# Autodesk Inventor assembly: Assembly1
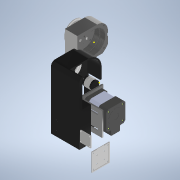
[picture p0: Inventor's stored thumbnail of the model, 180x180]
Saved by Autodesk Inventor 2022 (Build 260153000, 153)
## iProperties
Created: 2022-03-19
Part Number: Assembly1
Document SubType Name: Assembly
Designer: Mlees
Author: Mlees
## Documents named in this file (18)
- C:\Users\Mlees\Desktop\504Engineering\Stepper-Servo_Based_Robotic_Arm\Designs\Documentation_assembly\Assembly1.iam
- C:\Users\Mlees\Desktop\504Engineering\Stepper-Servo_Based_Robotic_Arm\Designs\Version_7\Created_Parts\Combined_Gear_Box_Modified_3.ipt
- C:\Users\Mlees\Desktop\504Engineering\Stepper-Servo_Based_Robotic_Arm\Designs\Version_7\Created_Parts\Metal_AttachmentBracket.ipt
- C:\Users\Mlees\Desktop\504Engineering\Stepper-Servo_Based_Robotic_Arm\Designs\Version_7\Downloaded_Parts\91290A113_Black-Oxide Alloy Steel Socket Head Screw.ipt
- C:\Users\Mlees\Desktop\504Engineering\Stepper-Servo_Based_Robotic_Arm\Designs\Version_7\Downloaded_Parts\nema17-speed-reducer-1.snapshot.9\Thread Insert M3 x 6mm v2.step.iam
- C:\Users\Mlees\Desktop\504Engineering\Stepper-Servo_Based_Robotic_Arm\Designs\Version_7\Downloaded_Parts\124125202-9-stp-mtr-17040w\stp-mtr-17040w.ipt
- C:\Users\Mlees\Desktop\504Engineering\Stepper-Servo_Based_Robotic_Arm\Designs\Version_7\Downloaded_Parts\GT2 20T Drive Pulley.ipt
- C:\Users\Mlees\Desktop\504Engineering\Stepper-Servo_Based_Robotic_Arm\Designs\Version_8\Downloaded_Parts\92010A018_Passivated 18-8 Stainless Steel Phillips Flat Head Screw.ipt
- C:\Users\Mlees\Desktop\504Engineering\Stepper-Servo_Based_Robotic_Arm\Designs\Version_8\Created_Parts\Belt_Bearing_Holder.ipt
- C:\Users\Mlees\Desktop\504Engineering\Stepper-Servo_Based_Robotic_Arm\Designs\Version_8\Created_Parts\Belt_Bearing_Holder_p2.ipt
- C:\Users\Mlees\Desktop\504Engineering\Stepper-Servo_Based_Robotic_Arm\Designs\Version_8\Downloaded_Parts\5972K225_Ball Bearing.ipt
- C:\Users\Mlees\Desktop\504Engineering\Stepper-Servo_Based_Robotic_Arm\Designs\Version_8\Downloaded_Parts\91290A059_Black-Oxide Alloy Steel Socket Head Screw_M3_30mm.ipt
- C:\Users\Mlees\Desktop\504Engineering\Stepper-Servo_Based_Robotic_Arm\Designs\Version_8\Downloaded_Parts\5972K327_Ball Bearing_6201-2Z.ipt
- C:\Users\Mlees\Desktop\504Engineering\Stepper-Servo_Based_Robotic_Arm\Designs\Version_8\Created_Parts\Combined_Gear_Box_Modified_2.ipt
- C:\Users\Mlees\Desktop\504Engineering\Stepper-Servo_Based_Robotic_Arm\Designs\Version_8\Created_Parts\Mag_Shield_Back.ipt
- C:\Users\Mlees\Desktop\504Engineering\Stepper-Servo_Based_Robotic_Arm\Designs\Version_8\Created_Parts\Mag_Sensor.ipt
- C:\Users\Mlees\Desktop\504Engineering\Stepper-Servo_Based_Robotic_Arm\Designs\Version_8\Downloaded_Parts\9403T15_Tight-Tolerance High-Strength 7075 Aluminum Rod.ipt
- C:\Users\Mlees\Desktop\504Engineering\Stepper-Servo_Based_Robotic_Arm\Designs\Version_8\Downloaded_Parts\GT2 60T Drive Pulley.ipt
## Components (29 placed, 17 different names)
1. Combined_Gear_Box_Modified_3:1 — Mate:1, Mate:2, Mate:3, Mate:4, Flush:1, Flush:2, Flush:3, Flush:4, Mate:5, Flush:5, Mate:6, Mate:15, Mate:16, Flush:6, Flush:7, Rotational:2, Rotational:3, Mate:27, Flush:12
2. Metal_AttachmentBracket:1 — Mate:5, Flush:5, Mate:6, Mate:11, Mate:12, Mate:13, Mate:14, Mate:17, Mate:18, Mate:19, Mate:20, Flush:8, Flush:9, Flush:10, Flush:11
3. 91290A113_Black-Oxide Alloy Steel Socket Head Screw:1 — Mate:7, Mate:12
4. 91290A113_Black-Oxide Alloy Steel Socket Head Screw:2 — Mate:8, Mate:11
5. 91290A113_Black-Oxide Alloy Steel Socket Head Screw:3 — Mate:9, Mate:13
6. 91290A113_Black-Oxide Alloy Steel Socket Head Screw:4 — Mate:10, Mate:14
7. Thread Insert M3 x 6mm v2.step:1 [sub-assembly] — Mate:1, Flush:3, Mate:8
8. Thread Insert M3 x 6mm v2.step:2 [sub-assembly] — Mate:4, Flush:1, Mate:9
9. Thread Insert M3 x 6mm v2.step:3 [sub-assembly] — Mate:3, Flush:4, Mate:10
10. Thread Insert M3 x 6mm v2.step:4 [sub-assembly] — Mate:2, Flush:2, Mate:7
11. Thread Insert M3 x 6mm v2.step:5 [sub-assembly] — Mate:15, Flush:6
12. Thread Insert M3 x 6mm v2.step:6 [sub-assembly] — Mate:16, Flush:7
13. stp-mtr-17040w:1 — Rotational:1
14. GT2 20T Drive Pulley:1 — Rotational:1
15. 92010A018_Passivated 18-8 Stainless Steel Phillips Flat Head Screw:1 — Mate:17, Flush:8
16. 92010A018_Passivated 18-8 Stainless Steel Phillips Flat Head Screw:2 — Mate:18, Flush:11
17. 92010A018_Passivated 18-8 Stainless Steel Phillips Flat Head Screw:3 — Mate:19, Flush:9
18. 92010A018_Passivated 18-8 Stainless Steel Phillips Flat Head Screw:4 — Mate:20, Flush:10
19. Belt_Bearing_Holder:1 — Mate:21, Mate:22, Mate:23, Mate:25, Rotational:3
20. Belt_Bearing_Holder_p2:1 — Mate:25, Mate:26
21. 5972K225_Ball Bearing:1 — Mate:21, Mate:23, Mate:24
22. 5972K225_Ball Bearing:2 — Mate:22, Mate:24, Mate:26
23. 91290A059_Black-Oxide Alloy Steel Socket Head Screw_M3_30mm:1 — Rotational:2
24. 5972K327_Ball Bearing_6201-2Z:1 — Mate:27, Flush:12
25. Combined_Gear_Box_Modified_2:1 — Mate:28, Mate:29
26. Mag_Shield_Back:1
27. Mag_Sensor:1
28. 9403T15_Tight-Tolerance High-Strength 7075 Aluminum Rod:1 — Rigid:1, Mate:28
29. GT2 60T Drive Pulley:1 — Rigid:1, Mate:29
## Relationships (45: Mate 29, Flush 12, RevoluteJoint 3, WeldJoint 1)
- Mate:1: Combined_Gear_Box_Modified_3:1 ↔ Thread Insert M3 x 6mm v2.step:1
- Mate:2: Combined_Gear_Box_Modified_3:1 ↔ Thread Insert M3 x 6mm v2.step:4
- Mate:3: Combined_Gear_Box_Modified_3:1 ↔ Thread Insert M3 x 6mm v2.step:3
- Mate:4: Combined_Gear_Box_Modified_3:1 ↔ Thread Insert M3 x 6mm v2.step:2
- Flush:1: Combined_Gear_Box_Modified_3:1 ↔ Thread Insert M3 x 6mm v2.step:2
- Flush:2: Combined_Gear_Box_Modified_3:1 ↔ Thread Insert M3 x 6mm v2.step:4
- Flush:3: Combined_Gear_Box_Modified_3:1 ↔ Thread Insert M3 x 6mm v2.step:1
- Flush:4: Combined_Gear_Box_Modified_3:1 ↔ Thread Insert M3 x 6mm v2.step:3
- Mate:5: Combined_Gear_Box_Modified_3:1 ↔ Metal_AttachmentBracket:1
- Flush:5: Combined_Gear_Box_Modified_3:1 ↔ Metal_AttachmentBracket:1
- Mate:6: Combined_Gear_Box_Modified_3:1 ↔ Metal_AttachmentBracket:1
- Mate:7: 91290A113_Black-Oxide Alloy Steel Socket Head Screw:1 ↔ Thread Insert M3 x 6mm v2.step:4
- Mate:8: 91290A113_Black-Oxide Alloy Steel Socket Head Screw:2 ↔ Thread Insert M3 x 6mm v2.step:1
- Mate:9: 91290A113_Black-Oxide Alloy Steel Socket Head Screw:3 ↔ Thread Insert M3 x 6mm v2.step:2
- Mate:10: 91290A113_Black-Oxide Alloy Steel Socket Head Screw:4 ↔ Thread Insert M3 x 6mm v2.step:3
- Mate:11: Metal_AttachmentBracket:1 ↔ 91290A113_Black-Oxide Alloy Steel Socket Head Screw:2
- Mate:12: Metal_AttachmentBracket:1 ↔ 91290A113_Black-Oxide Alloy Steel Socket Head Screw:1
- Mate:13: Metal_AttachmentBracket:1 ↔ 91290A113_Black-Oxide Alloy Steel Socket Head Screw:3
- Mate:14: Metal_AttachmentBracket:1 ↔ 91290A113_Black-Oxide Alloy Steel Socket Head Screw:4
- Mate:15: Combined_Gear_Box_Modified_3:1 ↔ Thread Insert M3 x 6mm v2.step:5
- Mate:16: Combined_Gear_Box_Modified_3:1 ↔ Thread Insert M3 x 6mm v2.step:6
- Flush:6: Combined_Gear_Box_Modified_3:1 ↔ Thread Insert M3 x 6mm v2.step:5
- Flush:7: Combined_Gear_Box_Modified_3:1 ↔ Thread Insert M3 x 6mm v2.step:6
- Rotational:1 [RevoluteJoint] (5 mm): stp-mtr-17040w:1 ↔ GT2 20T Drive Pulley:1
- Mate:17: Metal_AttachmentBracket:1 ↔ 92010A018_Passivated 18-8 Stainless Steel Phillips Flat Head Screw:1
- Mate:18: Metal_AttachmentBracket:1 ↔ 92010A018_Passivated 18-8 Stainless Steel Phillips Flat Head Screw:2
- Mate:19: Metal_AttachmentBracket:1 ↔ 92010A018_Passivated 18-8 Stainless Steel Phillips Flat Head Screw:3
- Mate:20: Metal_AttachmentBracket:1 ↔ 92010A018_Passivated 18-8 Stainless Steel Phillips Flat Head Screw:4
- Flush:8 (-1 mm): Metal_AttachmentBracket:1 ↔ 92010A018_Passivated 18-8 Stainless Steel Phillips Flat Head Screw:1
- Flush:9 (-1 mm): Metal_AttachmentBracket:1 ↔ 92010A018_Passivated 18-8 Stainless Steel Phillips Flat Head Screw:3
- Flush:10 (-1 mm): Metal_AttachmentBracket:1 ↔ 92010A018_Passivated 18-8 Stainless Steel Phillips Flat Head Screw:4
- Flush:11 (-1 mm): Metal_AttachmentBracket:1 ↔ 92010A018_Passivated 18-8 Stainless Steel Phillips Flat Head Screw:2
- Mate:21: Belt_Bearing_Holder:1 ↔ 5972K225_Ball Bearing:1
- Mate:22: Belt_Bearing_Holder:1 ↔ 5972K225_Ball Bearing:2
- Mate:23: Belt_Bearing_Holder:1 ↔ 5972K225_Ball Bearing:1
- Mate:24: 5972K225_Ball Bearing:1 ↔ 5972K225_Ball Bearing:2
- Mate:25: Belt_Bearing_Holder:1 ↔ Belt_Bearing_Holder_p2:1
- Mate:26: Belt_Bearing_Holder_p2:1 ↔ 5972K225_Ball Bearing:2
- Rotational:2 [RevoluteJoint]: Combined_Gear_Box_Modified_3:1 ↔ 91290A059_Black-Oxide Alloy Steel Socket Head Screw_M3_30mm:1
- Rotational:3 [RevoluteJoint] (6 mm): Combined_Gear_Box_Modified_3:1 ↔ Belt_Bearing_Holder:1
- Mate:27: Combined_Gear_Box_Modified_3:1 ↔ 5972K327_Ball Bearing_6201-2Z:1
- Flush:12 (-2 mm): Combined_Gear_Box_Modified_3:1 ↔ 5972K327_Ball Bearing_6201-2Z:1
- Rigid:1 [WeldJoint]: 9403T15_Tight-Tolerance High-Strength 7075 Aluminum Rod:1 ↔ GT2 60T Drive Pulley:1
- Mate:28: Combined_Gear_Box_Modified_2:1 ↔ 9403T15_Tight-Tolerance High-Strength 7075 Aluminum Rod:1
- Mate:29: Combined_Gear_Box_Modified_2:1 ↔ GT2 60T Drive Pulley:1
